# Autodesk Inventor assembly: DesignVer_2
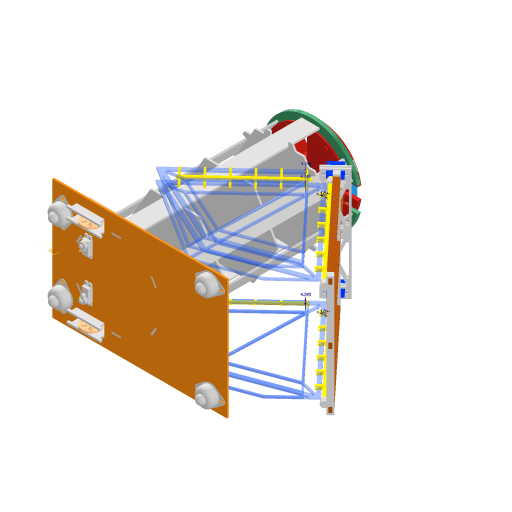
[picture p0: Inventor's stored thumbnail of the model, 512x512]
Saved by Autodesk Inventor 2024 (Build 280153000, 153)
## iProperties
Created: 2024-04-09
Part Number: DesignVer_2
Document SubType Name: Assembly
Designer: USER
Author: USER
## Documents named in this file (19)
- E:\university\大三\大三下\機工實務\圖檔\DesignVer2_encoder_MG996\DesignVer_2.iam
- E:\university\大三\大三下\機工實務\圖檔\DesignVer2_encoder_MG996\cow_wheel.ipt
- E:\university\大三\大三下\機工實務\圖檔\DesignVer2_encoder_MG996\back_down_hold.ipt
- E:\university\大三\大三下\機工實務\圖檔\DesignVer2_encoder_MG996\middle_space.ipt
- E:\university\大三\大三下\機工實務\圖檔\DesignVer2_encoder_MG996\rolling_plate.ipt
- E:\university\大三\大三下\機工實務\圖檔\DesignVer2_encoder_MG996\rolling_plate_top.ipt
- E:\university\大三\大三下\機工實務\圖檔\DesignVer2_encoder_MG996\rolling_plate_small.ipt
- E:\university\大三\大三下\機工實務\圖檔\DesignVer2_encoder_MG996\左右.ipt
- E:\university\大三\大三下\機工實務\圖檔\DesignVer2_encoder_MG996\左右2.ipt
- E:\university\大三\大三下\機工實務\圖檔\DesignVer2_encoder_MG996\馬達.ipt
- E:\university\大三\大三下\機工實務\圖檔\DesignVer2_encoder_MG996\軸.ipt
- E:\university\大三\大三下\機工實務\圖檔\DesignVer2_encoder_MG996\螺絲.ipt
- E:\university\大三\大三下\機工實務\圖檔\DesignVer2_encoder_MG996\sail.iam
- E:\university\大三\大三下\機工實務\圖檔\DesignVer2_encoder_MG996\Base_final.ipt
- E:\university\大三\大三下\機工實務\圖檔\DesignVer2_encoder_MG996\[3DP]back_cir_hold_final.ipt
- E:\university\大三\大三下\機工實務\圖檔\DesignVer2_encoder_MG996\MG996R\MG_996R.iam
- E:\university\大三\大三下\機工實務\圖檔\DesignVer2_encoder_MG996\middle_space_3.ipt
- E:\university\大三\大三下\機工實務\圖檔\encoder\encoder.iam
- E:\university\大三\大三下\機工實務\圖檔\DesignVer2_encoder_MG996\Servo Motor SG90.ipt
## Components (34 placed, 18 different names)
1. cow_wheel:3 — 貼合:80, 貼合:81, 貼合:85
2. cow_wheel:4 — 貼合:75, 貼合:76, 貼合:77, 貼合:78, 貼合:79
3. back_down_hold:1 — 貼合:99, 貼合:100, 貼合:101, 貼合:102, 貼合:107
4. back_down_hold:2 — 齊平:14, 相切:1, 齊平:28, 貼合:92, 貼合:93, 貼合:94
5. back_down_hold:3 — 齊平:5, 貼合:47, 齊平:13, 貼合:90, 貼合:91, 貼合:108, 貼合:138, 貼合:139, 貼合:140
6. back_down_hold:4 — 貼合:87, 貼合:97, 貼合:98
7. back_down_hold:5 — 齊平:6, 貼合:46, 齊平:12, 貼合:48, 貼合:88, 貼合:89, 貼合:105
8. back_down_hold:6 — 齊平:5, 齊平:6, 貼合:95, 貼合:96, 貼合:109
9. middle_space:1 — 齊平:13, 貼合:48, 齊平:14, 齊平:28
10. middle_space:2 — 貼合:46, 齊平:12, 貼合:47
11. rolling_plate:1 — 貼合:49, 貼合:50, 齊平:15, 貼合:55, 齊平:22, 齊平:23
12. rolling_plate:2 — 貼合:56, 貼合:57, 齊平:24, 貼合:110
13. rolling_plate_top:1 — 貼合:49, 貼合:50, 齊平:15, 相切:1, 貼合:58, 貼合:59, 貼合:60, 貼合:61, 貼合:62, 貼合:63
14. rolling_plate_small:1 — 貼合:52, 齊平:16, 齊平:19, 貼合:56, 齊平:24, 貼合:142, 貼合:143, 貼合:144
15. rolling_plate_small:2 — 貼合:52, 貼合:53, 齊平:16, 齊平:17, 齊平:19, 齊平:20, 貼合:57
16. rolling_plate_small:3 — 貼合:53, 貼合:54, 齊平:17, 齊平:18, 齊平:20, 齊平:21
17. rolling_plate_small:4 — 貼合:54, 齊平:18, 齊平:21, 貼合:55, 齊平:22, 齊平:23
18. 左右:1 — 貼合:58, 貼合:59, 貼合:60, 貼合:66, 貼合:67, 齊平:26, 貼合:68, 齊平:27
19. 左右2:1 — 貼合:61, 貼合:62, 貼合:63, 貼合:74
20. 馬達:1 — 貼合:64, 貼合:65, 貼合:69, 貼合:70, 貼合:71
21. 軸:1 — 貼合:64, 貼合:65, 貼合:73, 貼合:106
22. 螺絲:1 — 齊平:25, 貼合:66, 貼合:67, 齊平:26, 貼合:69, 貼合:70
23. 螺絲:2 — 齊平:25, 貼合:68, 齊平:27, 貼合:71
24. sail:1 [sub-assembly] — 貼合:73, 貼合:74, 貼合:106
25. Base_final:1 — 貼合:75, 貼合:76, 貼合:77, 貼合:78, 貼合:79, 貼合:80, 貼合:81, 貼合:85, 貼合:87, 貼合:88, 貼合:89, 貼合:90, 貼合:91, 貼合:92, 貼合:93, 貼合:94, 貼合:95, 貼合:96, 貼合:97, 貼合:98, 貼合:99, 貼合:100, 貼合:101, 貼合:102, 貼合:105, 貼合:115, 貼合:116, 貼合:117, 貼合:118, 貼合:131, 貼合:134, 角度:2, 角度:4, 齊平:29, 貼合:145, 貼合:146, 貼合:147, 貼合:148, 貼合:149, 貼合:151, 貼合:152, 貼合:153, 角度:5, 齊平:33, 齊平:34, 齊平:35, 齊平:36, 貼合:154
26. [3DP]back_cir_hold_final:1 — 貼合:107, 貼合:108, 貼合:109, 貼合:110, 貼合:142
27. cow_wheel:5 — 貼合:131, 貼合:145, 貼合:146, 貼合:147
28. cow_wheel:6 — 貼合:134, 貼合:148, 貼合:149
29. MG_996R:1 [sub-assembly] — 角度:2, 貼合:141, 貼合:143, 貼合:144
30. middle_space_3:1 — 貼合:138, 貼合:139, 貼合:140, 貼合:141
31. encoder:1 [sub-assembly] — 角度:3, 角度:4, 齊平:30, 貼合:151, 齊平:31, 貼合:154
32. encoder:2 [sub-assembly] — 角度:3, 齊平:29, 齊平:30, 齊平:31, 貼合:152
33. Servo Motor SG90:1 — 齊平:32, 貼合:153, 角度:5, 齊平:33, 齊平:34
34. Servo Motor SG90:2 — 齊平:32, 齊平:35, 齊平:36
## Relationships (113: Mate 81, Flush 27, Angle 4, Tangent 1)
- 齊平:5 [Flush]: back_down_hold:3 ↔ back_down_hold:6
- 齊平:6 [Flush]: back_down_hold:5 ↔ back_down_hold:6
- 貼合:46 [Mate]: back_down_hold:5 ↔ middle_space:2
- 齊平:12 [Flush]: back_down_hold:5 ↔ middle_space:2
- 貼合:47 [Mate]: back_down_hold:3 ↔ middle_space:2
- 齊平:13 [Flush]: back_down_hold:3 ↔ middle_space:1
- 貼合:48 [Mate]: back_down_hold:5 ↔ middle_space:1
- 齊平:14 [Flush]: back_down_hold:2 ↔ middle_space:1
- 貼合:49 [Mate]: rolling_plate:1 ↔ rolling_plate_top:1
- 貼合:50 [Mate]: rolling_plate:1 ↔ rolling_plate_top:1
- 齊平:15 [Flush]: rolling_plate:1 ↔ rolling_plate_top:1
- 相切:1 [Tangent]: back_down_hold:2 ↔ rolling_plate_top:1
- 貼合:52 [Mate]: rolling_plate_small:1 ↔ rolling_plate_small:2
- 貼合:53 [Mate]: rolling_plate_small:2 ↔ rolling_plate_small:3
- 貼合:54 [Mate]: rolling_plate_small:3 ↔ rolling_plate_small:4
- 齊平:16 [Flush]: rolling_plate_small:1 ↔ rolling_plate_small:2
- 齊平:17 [Flush]: rolling_plate_small:2 ↔ rolling_plate_small:3
- 齊平:18 [Flush]: rolling_plate_small:3 ↔ rolling_plate_small:4
- 齊平:19 [Flush]: rolling_plate_small:1 ↔ rolling_plate_small:2
- 齊平:20 [Flush]: rolling_plate_small:2 ↔ rolling_plate_small:3
- 齊平:21 [Flush]: rolling_plate_small:3 ↔ rolling_plate_small:4
- 貼合:55 [Mate]: rolling_plate:1 ↔ rolling_plate_small:4
- 齊平:22 [Flush]: rolling_plate:1 ↔ rolling_plate_small:4
- 齊平:23 [Flush]: rolling_plate:1 ↔ rolling_plate_small:4
- 貼合:56 [Mate]: rolling_plate:2 ↔ rolling_plate_small:1
- 貼合:57 [Mate]: rolling_plate:2 ↔ rolling_plate_small:2
- 齊平:24 [Flush]: rolling_plate:2 ↔ rolling_plate_small:1
- 貼合:58 [Mate]: rolling_plate_top:1 ↔ 左右:1
- 貼合:59 [Mate]: rolling_plate_top:1 ↔ 左右:1
- 貼合:60 [Mate]: rolling_plate_top:1 ↔ 左右:1
- 貼合:61 [Mate]: rolling_plate_top:1 ↔ 左右2:1
- 貼合:62 [Mate]: rolling_plate_top:1 ↔ 左右2:1
- 貼合:63 [Mate]: rolling_plate_top:1 ↔ 左右2:1
- 貼合:64 [Mate]: 馬達:1 ↔ 軸:1
- 貼合:65 [Mate]: 馬達:1 ↔ 軸:1
- 齊平:25 [Flush]: 螺絲:1 ↔ 螺絲:2
- 貼合:66 [Mate]: 左右:1 ↔ 螺絲:1
- 貼合:67 [Mate]: 左右:1 ↔ 螺絲:1
- 齊平:26 [Flush]: 左右:1 ↔ 螺絲:1
- 貼合:68 [Mate]: 左右:1 ↔ 螺絲:2
- 齊平:27 [Flush]: 左右:1 ↔ 螺絲:2
- 貼合:69 [Mate]: 馬達:1 ↔ 螺絲:1
- 貼合:70 [Mate]: 馬達:1 ↔ 螺絲:1
- 貼合:71 [Mate]: 馬達:1 ↔ 螺絲:2
- 齊平:28 [Flush]: back_down_hold:2 ↔ middle_space:1
- 貼合:73 [Mate]: 軸:1 ↔ sail:1
- 貼合:74 [Mate] (0.1 mm): 左右2:1 ↔ sail:1
- 貼合:75 [Mate]: cow_wheel:4 ↔ Base_final:1
- 貼合:76 [Mate]: cow_wheel:4 ↔ Base_final:1
- 貼合:77 [Mate]: cow_wheel:4 ↔ Base_final:1
- 貼合:78 [Mate]: cow_wheel:4 ↔ Base_final:1
- 貼合:79 [Mate]: cow_wheel:4 ↔ Base_final:1
- 貼合:80 [Mate]: cow_wheel:3 ↔ Base_final:1
- 貼合:81 [Mate]: cow_wheel:3 ↔ Base_final:1
- 貼合:85 [Mate]: cow_wheel:3 ↔ Base_final:1
- 貼合:87 [Mate]: back_down_hold:4 ↔ Base_final:1
- 貼合:88 [Mate]: back_down_hold:5 ↔ Base_final:1
- 貼合:89 [Mate]: back_down_hold:5 ↔ Base_final:1
- 貼合:90 [Mate]: back_down_hold:3 ↔ Base_final:1
- 貼合:91 [Mate]: back_down_hold:3 ↔ Base_final:1
- 貼合:92 [Mate]: back_down_hold:2 ↔ Base_final:1
- 貼合:93 [Mate]: back_down_hold:2 ↔ Base_final:1
- 貼合:94 [Mate]: back_down_hold:2 ↔ Base_final:1
- 貼合:95 [Mate]: back_down_hold:6 ↔ Base_final:1
- 貼合:96 [Mate]: back_down_hold:6 ↔ Base_final:1
- 貼合:97 [Mate]: back_down_hold:4 ↔ Base_final:1
- 貼合:98 [Mate]: back_down_hold:4 ↔ Base_final:1
- 貼合:99 [Mate]: back_down_hold:1 ↔ Base_final:1
- 貼合:100 [Mate]: back_down_hold:1 ↔ Base_final:1
- 貼合:101 [Mate]: back_down_hold:1 ↔ Base_final:1
- 貼合:102 [Mate]: back_down_hold:1 ↔ Base_final:1
- 貼合:105 [Mate]: back_down_hold:5 ↔ Base_final:1
- 貼合:106 [Mate]: 軸:1 ↔ sail:1
- 貼合:107 [Mate]: back_down_hold:1 ↔ [3DP]back_cir_hold_final:1
- 貼合:108 [Mate]: back_down_hold:3 ↔ [3DP]back_cir_hold_final:1
- 貼合:109 [Mate]: back_down_hold:6 ↔ [3DP]back_cir_hold_final:1
- 貼合:110 [Mate] (0.5 mm): rolling_plate:2 ↔ [3DP]back_cir_hold_final:1
- 貼合:115 [Mate]: Base_final:1
- 貼合:116 [Mate]: Base_final:1
- 貼合:117 [Mate]: Base_final:1
- 貼合:118 [Mate]: Base_final:1
- 貼合:119 [Mate]
- 貼合:120 [Mate]
- 貼合:131 [Mate]: Base_final:1 ↔ cow_wheel:5
- 貼合:134 [Mate]: Base_final:1 ↔ cow_wheel:6
- 角度:2 [Angle] (0 deg): Base_final:1 ↔ MG_996R:1
- 貼合:138 [Mate]: back_down_hold:3 ↔ middle_space_3:1
- 貼合:139 [Mate]: back_down_hold:3 ↔ middle_space_3:1
- 貼合:140 [Mate]: back_down_hold:3 ↔ middle_space_3:1
- 貼合:141 [Mate]: MG_996R:1 ↔ middle_space_3:1
- 貼合:142 [Mate]: rolling_plate_small:1 ↔ [3DP]back_cir_hold_final:1
- 貼合:143 [Mate]: rolling_plate_small:1 ↔ MG_996R:1
- 貼合:144 [Mate]: rolling_plate_small:1 ↔ MG_996R:1
- 角度:3 [Angle] (0 deg): encoder:1 ↔ encoder:2
- 角度:4 [Angle] (0 deg): Base_final:1 ↔ encoder:1
- 齊平:29 [Flush] (-12 mm): Base_final:1 ↔ encoder:2
- 齊平:30 [Flush]: encoder:1 ↔ encoder:2
- 貼合:145 [Mate]: Base_final:1 ↔ cow_wheel:5
- 貼合:146 [Mate]: Base_final:1 ↔ cow_wheel:5
- 貼合:147 [Mate]: Base_final:1 ↔ cow_wheel:5
- 貼合:148 [Mate]: Base_final:1 ↔ cow_wheel:6
- 貼合:149 [Mate]: Base_final:1 ↔ cow_wheel:6
- 貼合:151 [Mate] (0.1 mm): Base_final:1 ↔ encoder:1
- 齊平:31 [Flush]: encoder:1 ↔ encoder:2
- 貼合:152 [Mate] (0.1 mm): Base_final:1 ↔ encoder:2
- 齊平:32 [Flush]: Servo Motor SG90:1 ↔ Servo Motor SG90:2
- 貼合:153 [Mate]: Base_final:1 ↔ Servo Motor SG90:1
- 角度:5 [Angle] (0 deg): Base_final:1 ↔ Servo Motor SG90:1
- 齊平:33 [Flush] (55 mm): Base_final:1 ↔ Servo Motor SG90:1
- 齊平:34 [Flush] (55 mm): Base_final:1 ↔ Servo Motor SG90:1
- 齊平:35 [Flush] (55 mm): Base_final:1 ↔ Servo Motor SG90:2
- 齊平:36 [Flush] (55 mm): Base_final:1 ↔ Servo Motor SG90:2
- 貼合:154 [Mate] (0.1 mm): Base_final:1 ↔ encoder:1
